# Autodesk Inventor assembly: Camera
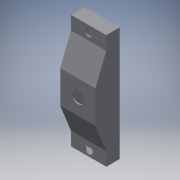
[picture p0: Inventor's stored thumbnail of the model, 180x180]
Saved by Autodesk Inventor 2016 (Build 200138000, 138)
## iProperties
Created: 2015-09-28
Part Number: Camera
Document SubType Name: Assembly
Designer: fei
Author: fei
## Documents named in this file (3)
- C:\Users\fei\Desktop\Robot_Head\Camera.iam
- C:\Users\fei\Desktop\Robot_Head\Cam_support.ipt
- C:\Users\fei\Desktop\Robot_Head\Up_cam_support.ipt
## Components (2 placed, 2 different names)
1. Cam_support:1 — Mate:1, Mate:2, Mate:3
2. Up_cam_support:1 — Mate:1, Mate:2, Mate:3
## Relationships (3: Mate 3)
- Mate:1: Cam_support:1 ↔ Up_cam_support:1
- Mate:2: Cam_support:1 ↔ Up_cam_support:1
- Mate:3: Cam_support:1 ↔ Up_cam_support:1
